# Autodesk Inventor assembly: motor
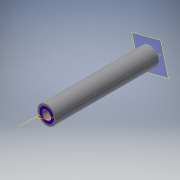
[picture p0: Inventor's stored thumbnail of the model, 180x180]
Saved by Autodesk Inventor 2016 SP1 (Build 200210100, 210)
## iProperties
Created: 2017-07-05
Part Number: motor
Material: Типовые
Document SubType Name: Assembly
Designer: user
Author: user
## Documents named in this file (6)
- D:\WORK\MOLOT\motor.iam
- D:\WORK\MOLOT\shtamp.ipt
- D:\WORK\MOLOT\tube.ipt
- D:\WORK\MOLOT\isolation.ipt
- D:\WORK\MOLOT\wire.ipt
- D:\WORK\MOLOT\tag.ipt
## Components (291 placed, 5 different names)
1. shtamp:1 — Совмещение:2, Совмещение:5, Совмещение:6
2. tube:1 — Совмещение:1
3. tag:1
4. isolation:1 — Совмещение:3, Совмещение:4, Касательность:1, Заподлицо:2
5. isolation:2
6. isolation:3
7. isolation:4
8. isolation:5
9. isolation:6
10. isolation:7
11. isolation:8
12. isolation:9
13. isolation:10
14. isolation:11
15. isolation:12
16. isolation:13
17. isolation:14
18. isolation:15
19. isolation:16
20. isolation:17
21. isolation:18
22. isolation:19
23. isolation:20
24. isolation:21
25. isolation:22
26. isolation:23
27. isolation:24
28. isolation:25
29. isolation:26
30. isolation:27
31. isolation:28
32. isolation:29
33. isolation:30
34. isolation:31
35. isolation:32
36. isolation:33
37. isolation:34
38. isolation:35
39. isolation:36
40. isolation:37
41. isolation:38
42. isolation:39
43. isolation:40
44. isolation:41
45. isolation:42
46. isolation:43
47. isolation:44
48. isolation:45
49. isolation:46
50. isolation:47
51. isolation:48
52. wire:1 — Совмещение:9, Касательность:1, Касательность:2, Заподлицо:2, Заподлицо:3, Совмещение:23
53. wire:2 — Совмещение:13, Касательность:2, Касательность:3, Заподлицо:3, Заподлицо:4
54. wire:3 — Совмещение:15, Касательность:3, Касательность:4, Заподлицо:4, Заподлицо:5
55. wire:4 — Совмещение:17, Касательность:4, Касательность:5, Заподлицо:5, Заподлицо:6
56. wire:5 — Совмещение:18, Касательность:5, Заподлицо:6
57. wire:6
58. wire:7
59. wire:8
60. wire:9
61. wire:10
62. wire:11
63. wire:12
64. wire:13
65. wire:14
66. wire:15
67. wire:16
68. wire:17
69. wire:18
70. wire:19
71. wire:20
72. wire:21
73. wire:22
74. wire:23
75. wire:24
76. wire:25
77. wire:26
78. wire:27
79. wire:28
80. wire:29
81. wire:30
82. wire:31
83. wire:32
84. wire:33
85. wire:34
86. wire:35
87. wire:36
88. wire:37
89. wire:38
90. wire:39
91. wire:40
92. wire:41
93. wire:42
94. wire:43
95. wire:44
96. wire:45
97. wire:46
98. wire:47
99. wire:48
100. wire:49
101. wire:50
102. wire:51
103. wire:52
104. wire:53
105. wire:54
106. wire:55
107. wire:56
108. wire:57
109. wire:58
110. wire:59
111. wire:60
112. wire:61
113. wire:62
114. wire:63
115. wire:64
116. wire:65
117. wire:66
118. wire:67
119. wire:68
120. wire:69
121. wire:70
122. wire:71
123. wire:72
124. wire:73
125. wire:74
126. wire:75
127. wire:76
128. wire:77
129. wire:78
130. wire:79
131. wire:80
132. wire:81
133. wire:82
134. wire:83
135. wire:84
136. wire:85
137. wire:86
138. wire:87
139. wire:88
140. wire:89
141. wire:90
142. wire:91
143. wire:92
144. wire:93
145. wire:94
146. wire:95
147. wire:96
148. wire:97
149. wire:98
150. wire:99
151. wire:100
152. wire:101
153. wire:102
154. wire:103
155. wire:104
156. wire:105
157. wire:106
158. wire:107
159. wire:108
160. wire:109
161. wire:110
162. wire:111
163. wire:112
164. wire:113
165. wire:114
166. wire:115
167. wire:116
168. wire:117
169. wire:118
170. wire:119
171. wire:120
172. wire:121
173. wire:122
174. wire:123
175. wire:124
176. wire:125
177. wire:126 — Совмещение:22
178. wire:127
179. wire:128
180. wire:129
181. wire:130
182. wire:131
183. wire:132
184. wire:133
185. wire:134
186. wire:135
187. wire:136
188. wire:137
189. wire:138
190. wire:139
191. wire:140
192. wire:141
193. wire:142
194. wire:143
195. wire:144
196. wire:145
197. wire:146
198. wire:147
199. wire:148
200. wire:149
201. wire:150
202. wire:151
203. wire:152
204. wire:153
205. wire:154
206. wire:155
207. wire:156
208. wire:157
209. wire:158
210. wire:159
211. wire:160
212. wire:161
213. wire:162
214. wire:163
215. wire:164
216. wire:165
217. wire:166
218. wire:167
219. wire:168
220. wire:169
221. wire:170
222. wire:171
223. wire:172
224. wire:173
225. wire:174
226. wire:175
227. wire:176
228. wire:177
229. wire:178
230. wire:179
231. wire:180
232. wire:181
233. wire:182
234. wire:183
235. wire:184
236. wire:185
237. wire:186
238. wire:187
239. wire:188
240. wire:189
241. wire:190
242. wire:191
243. wire:192
244. wire:193
245. wire:194
246. wire:195
247. wire:196
248. wire:197
249. wire:198
250. wire:199
251. wire:200
252. wire:201
253. wire:202
254. wire:203
255. wire:204
256. wire:205
257. wire:206
258. wire:207
259. wire:208
260. wire:209
261. wire:210
262. wire:211
263. wire:212
264. wire:213
265. wire:214
266. wire:215
267. wire:216
268. wire:217
269. wire:218
270. wire:219
271. wire:220
272. wire:221
273. wire:222
274. wire:223
275. wire:224
276. wire:225
277. wire:226
278. wire:227
279. wire:228
280. wire:229
281. wire:230
282. wire:231
283. wire:232
284. wire:233
285. wire:234
286. wire:235
287. wire:236
288. wire:237
289. wire:238
290. wire:239
291. wire:240
## Component patterns: (48 elements, first: isolation:1), (48 elements, first: wire:1 + wire:2 + wire:3 + wire:4 + wire:5)
## Relationships (34: Mate 24, Tangent 5, Flush 5)
- Совмещение:1 [Mate]: tube:1
- Совмещение:2 [Mate]: shtamp:1
- Совмещение:3 [Mate]: isolation:1
- Совмещение:4 [Mate]: isolation:1
- Совмещение:5 [Mate]: shtamp:1
- Совмещение:6 [Mate]: shtamp:1
- Совмещение:7 [Mate]
- Совмещение:8 [Mate]
- Совмещение:9 [Mate]: wire:1
- Совмещение:10 [Mate]
- Совмещение:11 [Mate]
- Совмещение:12 [Mate]
- Касательность:1 [Tangent]: isolation:1 ↔ wire:1
- Совмещение:13 [Mate]: wire:2
- Совмещение:14 [Mate]
- Касательность:2 [Tangent]: wire:1 ↔ wire:2
- Совмещение:15 [Mate]: wire:3
- Совмещение:16 [Mate]
- Касательность:3 [Tangent]: wire:2 ↔ wire:3
- Совмещение:17 [Mate]: wire:4
- Совмещение:18 [Mate]: wire:5
- Совмещение:20 [Mate]
- Касательность:4 [Tangent]: wire:3 ↔ wire:4
- Совмещение:21 [Mate]
- Касательность:5 [Tangent]: wire:4 ↔ wire:5
- Заподлицо:2 [Flush]: isolation:1 ↔ wire:1
- Заподлицо:3 [Flush]: wire:1 ↔ wire:2
- Заподлицо:4 [Flush]: wire:2 ↔ wire:3
- Заподлицо:5 [Flush]: wire:3 ↔ wire:4
- Заподлицо:6 [Flush]: wire:4 ↔ wire:5
- Совмещение:22 [Mate]: wire:126
- Совмещение:23 [Mate]: wire:1
- Совмещение:24 [Mate]
- Совмещение:25 [Mate]
